# Autodesk Inventor assembly: BoyaEnsamble
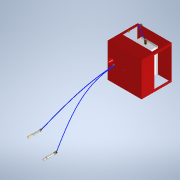
[picture p0: Inventor's stored thumbnail of the model, 180x180]
Saved by Autodesk Inventor 2020 (Build 240168000, 168)
## iProperties
Created: 2021-10-16
Part Number: BoyaEnsamble
Document SubType Name: Assembly
Designer: DANIEL
Mass: 28533.1 g
Surface Area: 26349.6 cm^2
Volume: 28533.1 cm^3
Density: 1 g/cm^3
Author: DANIEL
## Documents named in this file (15)
- C:\Users\DANIEL\Documents\Personal\Convocatorias\Escollera\tesis\CAD\V3\BoyaEnsamble.iam
- C:\Users\DANIEL\Documents\Personal\Convocatorias\Escollera\tesis\CAD\V3\CajaBoya.ipt
- C:\Users\DANIEL\Documents\Personal\Convocatorias\Escollera\tesis\CAD\V3\cajaEléctrica.ipt
- C:\Users\DANIEL\Documents\Personal\Convocatorias\Escollera\tesis\CAD\V3\W520.iam
- C:\Users\DANIEL\Documents\Personal\Convocatorias\Escollera\tesis\CAD\V3\techo.ipt
- C:\Users\DANIEL\Documents\Personal\Convocatorias\Escollera\tesis\CAD\V3\EnsamblajeCircuito.iam
- C:\Users\DANIEL\Documents\Personal\Convocatorias\Escollera\tesis\CAD\V3\antena.ipt
- C:\Users\DANIEL\Documents\Personal\Convocatorias\Escollera\tesis\CAD\V3\BoyaEnsamble\AIP\Tubos y tuberías\Cable y arnés\BoyaEnsamble.Arnés2.iam
- C:\Users\DANIEL\Documents\Personal\Convocatorias\Escollera\tesis\CAD\V3\W504.ipt
- C:\Users\DANIEL\Documents\Personal\Convocatorias\Escollera\tesis\CAD\V3\packBaterias.iam
- C:\Users\DANIEL\Documents\Personal\Convocatorias\Escollera\tesis\CAD\V3\BoyaEnsamble\AIP\Tubos y tuberías\Cable y arnés\BoyaEnsamble.Arnés3.iam
- C:\Users\DANIEL\Documents\Personal\Convocatorias\Escollera\tesis\CAD\V3\BoyaEnsamble\AIP\Tubos y tuberías\Cable y arnés\BoyaEnsamble.Arnés4.iam
- C:\Users\DANIEL\Documents\Personal\Convocatorias\Escollera\tesis\CAD\V3\panelSolar.ipt
- C:\Users\DANIEL\Documents\Personal\Convocatorias\Escollera\tesis\CAD\V3\EnsamblajeCajaElectricaCompletaV3.iam
- C:\Users\DANIEL\Documents\Personal\Convocatorias\Escollera\tesis\CAD\V3\BoyaEnsamble\AIP\Tubos y tuberías\Cable y arnés\BoyaEnsamble.Arnés5.iam
## Components (14 placed, 14 different names)
1. CajaBoya:1 — Coincidencia:1, Coincidencia:2, Coincidencia:3, Coincidencia:4, Coincidencia:5, Coincidencia:6
2. cajaEléctrica:1 — Coincidencia:1, Coincidencia:2
3. W520:1 [sub-assembly] — Coincidencia:3
4. techo:1
5. EnsamblajeCircuito:1 [sub-assembly]
6. antena:1
7. Arnés2 [sub-assembly]
8. W504:1
9. packBaterias:1 [sub-assembly]
10. Arnés3 [sub-assembly]
11. Arnés4 [sub-assembly]
12. panelSolar:1 — Coincidencia:4
13. EnsamblajeCajaElectricaCompletaV3:1 [sub-assembly] — Coincidencia:5, Coincidencia:6
14. Arnés5 [sub-assembly]
## Relationships (6: Mate 6)
- Coincidencia:1 [Mate]: CajaBoya:1 ↔ cajaEléctrica:1
- Coincidencia:2 [Mate]: CajaBoya:1 ↔ cajaEléctrica:1
- Coincidencia:3 [Mate] (1000 mm): CajaBoya:1 ↔ W520:1
- Coincidencia:4 [Mate]: CajaBoya:1 ↔ panelSolar:1
- Coincidencia:5 [Mate]: CajaBoya:1 ↔ EnsamblajeCajaElectricaCompletaV3:1
- Coincidencia:6 [Mate]: CajaBoya:1 ↔ EnsamblajeCajaElectricaCompletaV3:1
